# Autodesk Inventor assembly: CompositeSupport
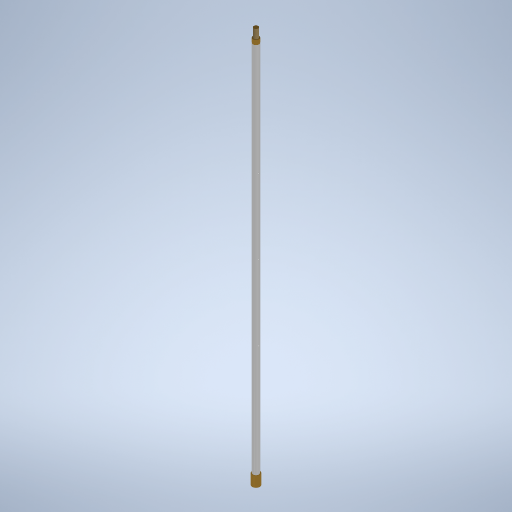
[picture p0: Inventor's stored thumbnail of the model, 512x512]
Saved by Autodesk Inventor 2024 (Build 280153000, 153)
## iProperties
Created: 2023-09-24
Part Number: CompositeSupport
Document SubType Name: Assembly
Designer: schanen
Author: schanen
## Documents named in this file (4)
- C:\Users\schanen\Documents\Inventor\he4inserts\CompositeSupport.iam
- C:\Users\schanen\Documents\Inventor\he4inserts\Fitting-1.ipt
- C:\Users\schanen\Documents\Inventor\he4inserts\Fitting-2.ipt
- C:\Users\schanen\Documents\Inventor\he4inserts\InsertTube6OD0.6W100L.ipt
## Components (3 placed, 3 different names)
1. Fitting-1:1 — Mate:1, Mate:3
2. Fitting-2:1 — Mate:2, Mate:4
3. InsertTube6OD0.6W100L:1 — Mate:1, Mate:2, Mate:3, Mate:4
## Relationships (4: Mate 4)
- Mate:1: Fitting-1:1 ↔ InsertTube6OD0.6W100L:1
- Mate:2: Fitting-2:1 ↔ InsertTube6OD0.6W100L:1
- Mate:3: Fitting-1:1 ↔ InsertTube6OD0.6W100L:1
- Mate:4: Fitting-2:1 ↔ InsertTube6OD0.6W100L:1
